# Autodesk Inventor assembly: Steel-Lock-Steel
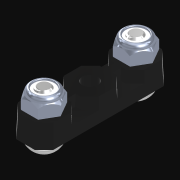
[picture p0: Inventor's stored thumbnail of the model, 180x180]
Saved by Autodesk Inventor 2021 (Build 250183000, 183)
## iProperties
Created: 2020-11-09
Part Number: Steel-Lock-Steel
Document SubType Name: Assembly
Designer: yuany
Author: yuany
## Documents named in this file (5)
- E:\VEX Cad\Assembly\KAUKAU\Premade Bearings\Steel-Lock-Steel.iam
- E:\VEX Cad\Library 1.2\Motion\Bearing Flat.ipt
- E:\VEX Cad\Library 1.2\Structure\Hardware\Nut Nylock.ipt
- E:\VEX Cad\Library 1.2\Structure\Hardware\Screw Steel - Hex\Screw 8-32 Steel .500.ipt
- E:\VEX Cad\Library 1.2\Structure\Hardware\Screw Steel - Hex.ipt
## Components (5 placed, 3 different names)
1. Bearing Flat:1 — Insert:1, Insert:2, Insert:3, Insert:4
2. Nut Nylock:1 — Insert:1
3. Screw 8-32 Steel .500:1 — Insert:4
4. Nut Nylock:2 — Insert:2
5. Screw 8-32 Steel .500:2 — Insert:3
## Relationships (4: Insert 4)
- Insert:1: Bearing Flat:1 ↔ Nut Nylock:1
- Insert:2: Bearing Flat:1 ↔ Nut Nylock:2
- Insert:3 (1.1684 mm): Bearing Flat:1 ↔ Screw 8-32 Steel .500:2
- Insert:4 (1.1684 mm): Bearing Flat:1 ↔ Screw 8-32 Steel .500:1
